# Autodesk Inventor assembly: Shaft Collar Metal
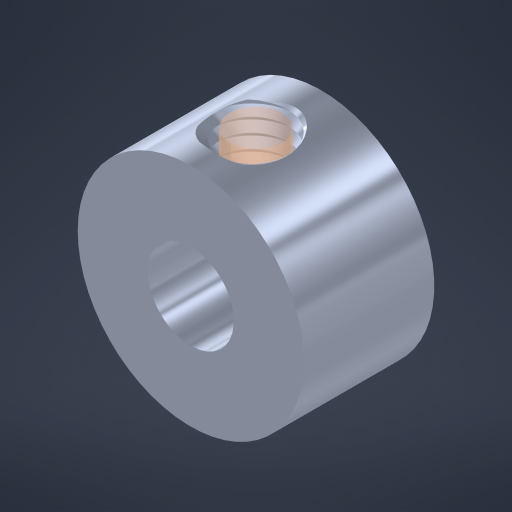
[picture p0: Inventor's stored thumbnail of the model, 512x512]
Saved by Autodesk Inventor 2023.2 (Build 272271000, 271)
## iProperties
Created: 2022-08-01
Part Number: Shaft Collar Metal
Document SubType Name: Assembly
Designer: ylu12
Author: ylu12
## Documents named in this file (3)
- D:\CAD\Parts\standard\Motion\Shafts\Shaft Collar\Shaft Collar No Screw.iam
- D:\CAD\Parts\standard\Motion\Shafts\Reference Parts\Shaft Collar Metal.ipt
- D:\CAD\Parts\standard\Motion\Shafts\Shaft Collar.iam
## Components (1 placed, 1 different names)
1. Shaft Collar Metal:1 — Mate:1, Mate:2, Flush:1
## Relationships (3: Mate 2, Flush 1)
- Mate:1: Shaft Collar Metal:1
- Mate:2: Shaft Collar Metal:1
- Flush:1: Shaft Collar Metal:1
